# Autodesk Inventor assembly: DERIVER_BALL_BEARING,REV_ENG
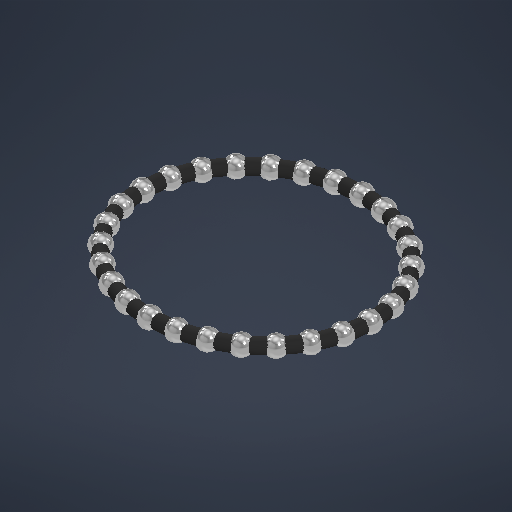
[picture p0: Inventor's stored thumbnail of the model, 512x512]
Saved by Autodesk Inventor 2026.2 (Build 302298010, 298A)
## iProperties
Created: 2026-03-06
Part Number: DERIVER_BALL_BEARING,REV_ENG
Document SubType Name: Assembly
Designer: 4aida
Author: 4aida
## Documents named in this file (3)
- C:\Users\4aida\OneDrive\Documents\GitHub\Design_II_Group6\REV_ENG\DERIVER_BALL_BEARING,REV_ENG.iam
- C:\Users\4aida\OneDrive\Documents\GitHub\Design_II_Group6\REV_ENG\2.5mm_BALL_BEARINGS.ipt
- C:\Users\4aida\OneDrive\Documents\GitHub\Design_II_Group6\REV_ENG\BEARING_SPACERS_CORE,REV-ENG.ipt
## Components (2 placed, 2 different names)
1. 2.5mm_BALL_BEARINGS:1 — Mate:3, Mate:4, Mate:5
2. BEARING_SPACERS_CORE,REV-ENG:1 — Mate:1, Mate:2, Flush:1
## Relationships (6: Mate 5, Flush 1)
- Mate:1: BEARING_SPACERS_CORE,REV-ENG:1
- Mate:2: BEARING_SPACERS_CORE,REV-ENG:1
- Flush:1: BEARING_SPACERS_CORE,REV-ENG:1
- Mate:3: 2.5mm_BALL_BEARINGS:1
- Mate:4: 2.5mm_BALL_BEARINGS:1
- Mate:5: 2.5mm_BALL_BEARINGS:1
